# Autodesk Inventor assembly: SimpleDesignV2 - 02
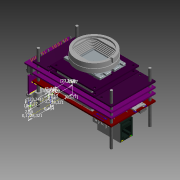
[picture p0: Inventor's stored thumbnail of the model, 180x180]
Saved by Autodesk Inventor 2015 (Build 190159000, 159)
## iProperties
Created: 2014-04-13
Part Number: SimpleDesignV2 - 02
Document SubType Name: Assembly
Designer: spichelh
Author: spichelh
## Documents named in this file (23)
- C:\Users\spichelh\Documents\GitHub\beta-hardware\Enclosure\SimpleDesign02\SimpleDesignV2 - 02.iam
- C:\Users\spichelh\Documents\GitHub\beta-hardware\Enclosure\SimpleDesign02\SFE-Host01.ipt
- C:\Users\spichelh\Documents\GitHub\beta-hardware\Enclosure\SimpleDesign02\SFE-ProcessingBoard01.ipt
- C:\Users\spichelh\Documents\GitHub\beta-hardware\Enclosure\SimpleDesign02\PCBModuleLeft02.ipt
- C:\Users\spichelh\Documents\GitHub\beta-hardware\Enclosure\SimpleDesign02\BetaBoard01.ipt
- C:\Users\spichelh\Documents\GitHub\beta-hardware\Enclosure\SimpleDesign02\PowerPCB01.ipt
- C:\Users\spichelh\Documents\GitHub\beta-hardware\Enclosure\SimpleDesign02\Samtec-PCIE-036-02-D-F-TH.ipt
- C:\Users\spichelh\Documents\GitHub\beta-hardware\Enclosure\SimpleDesign02\SensorCooler01.ipt
- C:\Users\spichelh\Documents\GitHub\beta-hardware\Enclosure\SimpleDesign02\CMV12000v1.ipt
- C:\Users\spichelh\Documents\GitHub\beta-hardware\Enclosure\SimpleDesign02\threaded-rod01.ipt
- C:\Users\spichelh\Documents\GitHub\beta-hardware\Enclosure\SimpleDesign02\Simple3DPrintEnclosure01.ipt
- C:\Users\spichelh\Documents\Inventor\Content Center Files\R2015\en-US\ANSI B18.6.4(04)\ANSI B18.6.4 - 4-24 - 0,375(1) B IA.ipt
- C:\Users\spichelh\Documents\GitHub\beta-hardware\Enclosure\SimpleDesign02\Simple3DPrintBackplate01.ipt
- C:\Users\spichelh\Documents\Inventor\Content Center Files\R2015\en-US\Nut GB_T 17880.1-1999\Nut GB_T 17880.1-1999 M3 x 7.5.ipt
- C:\Users\spichelh\Documents\GitHub\beta-hardware\Enclosure\SimpleDesign02\CoolingFan50x50-V01.ipt
- C:\Users\spichelh\Documents\Inventor\Content Center Files\R2015\en-US\ANSI B18.6.3(00)\ANSI B18.6.3 - 4-40 UNC - 0,125(32).ipt
- C:\Users\spichelh\Documents\GitHub\beta-hardware\Enclosure\SimpleDesign02\Sensormount_CMV12000.iam
- C:\Users\spichelh\Documents\GitHub\beta-hardware\Enclosure\SimpleDesign02\Sensormount_CMV12000_CNC.ipt
- C:\Users\spichelh\Documents\GitHub\beta-hardware\Enclosure\SimpleDesign02\footplate.ipt
- C:\Users\spichelh\Documents\GitHub\beta-hardware\Enclosure\SimpleDesign02\E Mount.ipt
- C:\Users\spichelh\Documents\GitHub\beta-hardware\Enclosure\SimpleDesign02\HDMI Plugin Module.ipt
- C:\Users\spichelh\Documents\GitHub\beta-hardware\Enclosure\SimpleDesign02\HDMIPluginModuleHolder02.ipt
- C:\Users\spichelh\Documents\GitHub\beta-hardware\Enclosure\SimpleDesign02\Zynq_Z010_uZed_F_Prod_simplified.ipt
## Components (37 placed, 22 different names)
1. SFE-Host01:1 — Mate:73, Flush:48, Flush:49, Flush:125, Flush:126, Mate:163
2. SFE-ProcessingBoard01:1 — Mate:73, Flush:48, Flush:49, Flush:109, Mate:134, Flush:112, Mate:136, Flush:123, Flush:124, Mate:159, Mate:209
3. PCBModuleLeft02:1 — Flush:109, Mate:134, Flush:113, Flush:114
4. BetaBoard01:1 — Mate:135, Flush:110, Flush:111, Flush:112, Mate:136, Flush:113, Flush:114, Mate:137, Mate:138, Flush:116, Mate:142, Mate:143, Flush:117, Mate:209
5. Zynq_Z010_uZed_F_Prod_simplified:1 — Mate:131, Flush:107, Flush:108, Mate:192, Mate:193, Mate:194, Mate:218
6. PowerPCB01:1 — Mate:131, Flush:107, Flush:108, Mate:135, Flush:110, Flush:111
7. Samtec-PCIE-036-02-D-F-TH:1 — Mate:137, Mate:138, Flush:116, Mate:219, Mate:221, Mate:222
8. Samtec-PCIE-036-02-D-F-TH:2 — Mate:142, Mate:143, Flush:117, Mate:213, Mate:214, Mate:215
9. SensorCooler01:1
10. PCBModuleLeft02:2 — Flush:123, Flush:124, Mate:159
11. CMV12000v1:1 — Flush:125, Flush:126, Mate:163, Mate:195, Flush:138, Mate:200, Mate:201
12. Sensormount_CMV12000_CNC:1 — Mate:195, Mate:196, Flush:137, Flush:138, Flush:139, Mate:197, Mate:198, Flush:140, Flush:141, Mate:199, Mate:200, Mate:201, Mate:202, Mate:203, Mate:204, Mate:205, Flush:146, Mate:206, Mate:208
13. threaded-rod01:1 — Mate:198, Flush:140
14. threaded-rod01:2 — Flush:139, Mate:197, Mate:217
15. threaded-rod01:3 — Mate:196, Flush:137, Mate:216
16. threaded-rod01:4 — Mate:177, Flush:141, Mate:199
17. Simple3DPrintEnclosure01:1 — Mate:173, Mate:174, Mate:175, Mate:176, Mate:185, Mate:186, Mate:187, Flush:133, Flush:134, Flush:135, Flush:136, Mate:202, Mate:203, Mate:204, Flush:142, Flush:143, Flush:144, Flush:145, Mate:210, Mate:211, Mate:212
18. Simple3DPrintBackplate01:1 — Mate:210, Mate:211, Mate:212
19. Cross Recessed 100° Flat Countersunk Head Tapping Screw - Type B - Type IA - Inch No. 4 - 24 -  3/8:1 — Mate:173, Flush:143
20. Cross Recessed 100° Flat Countersunk Head Tapping Screw - Type B - Type IA - Inch No. 4 - 24 -  3/8:2 — Mate:174, Flush:142
21. Cross Recessed 100° Flat Countersunk Head Tapping Screw - Type B - Type IA - Inch No. 4 - 24 -  3/8:3 — Mate:175, Flush:145
22. Cross Recessed 100° Flat Countersunk Head Tapping Screw - Type B - Type IA - Inch No. 4 - 24 -  3/8:4 — Mate:176, Flush:144
23. Nut GB/T 17880.1-1999 M3 x 7.5:1 — Mate:177
24. Nut GB/T 17880.1-1999 M3 x 7.5:2
25. Nut GB/T 17880.1-1999 M3 x 7.5:3
26. Nut GB/T 17880.1-1999 M3 x 7.5:4
27. CoolingFan50x50-V01:1 — Mate:185, Mate:186, Mate:187, Mate:188, Mate:189, Mate:190, Mate:191
28. Cross Recessed 100° Flat Countersunk Head Machine Screw - Type I - Inch 4-40 UNC x 0,125:1 — Mate:188, Flush:135
29. Cross Recessed 100° Flat Countersunk Head Machine Screw - Type I - Inch 4-40 UNC x 0,125:2 — Mate:189, Flush:133
30. Cross Recessed 100° Flat Countersunk Head Machine Screw - Type I - Inch 4-40 UNC x 0,125:3 — Mate:190, Flush:134
31. Cross Recessed 100° Flat Countersunk Head Machine Screw - Type I - Inch 4-40 UNC x 0,125:4 — Mate:191, Flush:136
32. Heatsink 31x31x10mm [sub-assembly] — Mate:192, Mate:193, Mate:194
33. footplate:1 — Mate:205, Flush:146, Mate:206, Mate:207
34. E Mount:1 — Mate:208
35. HDMIPluginModuleHolder02:1 — Mate:216, Mate:217, Mate:218
36. HDMI Plugin Module:1 — Mate:213, Mate:214, Mate:215
37. HDMI Plugin Module:2 — Mate:219, Mate:221, Mate:222
## Relationships (83: Mate 53, Flush 30)
- Mate:73: SFE-Host01:1 ↔ SFE-ProcessingBoard01:1
- Flush:48: SFE-Host01:1 ↔ SFE-ProcessingBoard01:1
- Flush:49: SFE-Host01:1 ↔ SFE-ProcessingBoard01:1
- Mate:131 (7 mm): Zynq_Z010_uZed_F_Prod_simplified:1 ↔ PowerPCB01:1
- Flush:107: Zynq_Z010_uZed_F_Prod_simplified:1 ↔ PowerPCB01:1
- Flush:108: Zynq_Z010_uZed_F_Prod_simplified:1 ↔ PowerPCB01:1
- Flush:109: SFE-ProcessingBoard01:1 ↔ PCBModuleLeft02:1
- Mate:134 (1 mm): SFE-ProcessingBoard01:1 ↔ PCBModuleLeft02:1
- Mate:135 (5 mm): BetaBoard01:1 ↔ PowerPCB01:1
- Flush:110: BetaBoard01:1 ↔ PowerPCB01:1
- Flush:111: BetaBoard01:1 ↔ PowerPCB01:1
- Flush:112: SFE-ProcessingBoard01:1 ↔ BetaBoard01:1
- Mate:136: SFE-ProcessingBoard01:1 ↔ BetaBoard01:1
- Flush:113: PCBModuleLeft02:1 ↔ BetaBoard01:1
- Flush:114: PCBModuleLeft02:1 ↔ BetaBoard01:1
- Mate:137: BetaBoard01:1 ↔ Samtec-PCIE-036-02-D-F-TH:1
- Mate:138: BetaBoard01:1 ↔ Samtec-PCIE-036-02-D-F-TH:1
- Flush:116 (1.4908 mm): BetaBoard01:1 ↔ Samtec-PCIE-036-02-D-F-TH:1
- Mate:142: BetaBoard01:1 ↔ Samtec-PCIE-036-02-D-F-TH:2
- Mate:143: BetaBoard01:1 ↔ Samtec-PCIE-036-02-D-F-TH:2
- Flush:117 (2.0906 mm): BetaBoard01:1 ↔ Samtec-PCIE-036-02-D-F-TH:2
- Flush:123: SFE-ProcessingBoard01:1 ↔ PCBModuleLeft02:2
- Flush:124: SFE-ProcessingBoard01:1 ↔ PCBModuleLeft02:2
- Mate:159 (2 mm): SFE-ProcessingBoard01:1 ↔ PCBModuleLeft02:2
- Flush:125 (11.875 mm): SFE-Host01:1 ↔ CMV12000v1:1
- Flush:126 (5.175 mm): SFE-Host01:1 ↔ CMV12000v1:1
- Mate:163 (3 mm): SFE-Host01:1 ↔ CMV12000v1:1
- Mate:173: Simple3DPrintEnclosure01:1 ↔ Cross Recessed 100° Flat Countersunk Head Tapping Screw - Type B - Type IA - Inch No. 4 - 24 -  3/8:1
- Mate:174: Simple3DPrintEnclosure01:1 ↔ Cross Recessed 100° Flat Countersunk Head Tapping Screw - Type B - Type IA - Inch No. 4 - 24 -  3/8:2
- Mate:175: Simple3DPrintEnclosure01:1 ↔ Cross Recessed 100° Flat Countersunk Head Tapping Screw - Type B - Type IA - Inch No. 4 - 24 -  3/8:3
- Mate:176: Simple3DPrintEnclosure01:1 ↔ Cross Recessed 100° Flat Countersunk Head Tapping Screw - Type B - Type IA - Inch No. 4 - 24 -  3/8:4
- Mate:177: threaded-rod01:4 ↔ Nut GB/T 17880.1-1999 M3 x 7.5:1
- Mate:185: Simple3DPrintEnclosure01:1 ↔ CoolingFan50x50-V01:1
- Mate:186: Simple3DPrintEnclosure01:1 ↔ CoolingFan50x50-V01:1
- Mate:187: Simple3DPrintEnclosure01:1 ↔ CoolingFan50x50-V01:1
- Mate:188: CoolingFan50x50-V01:1 ↔ Cross Recessed 100° Flat Countersunk Head Machine Screw - Type I - Inch 4-40 UNC x 0,125:1
- Mate:189: CoolingFan50x50-V01:1 ↔ Cross Recessed 100° Flat Countersunk Head Machine Screw - Type I - Inch 4-40 UNC x 0,125:2
- Mate:190: CoolingFan50x50-V01:1 ↔ Cross Recessed 100° Flat Countersunk Head Machine Screw - Type I - Inch 4-40 UNC x 0,125:3
- Mate:191: CoolingFan50x50-V01:1 ↔ Cross Recessed 100° Flat Countersunk Head Machine Screw - Type I - Inch 4-40 UNC x 0,125:4
- Flush:133: Simple3DPrintEnclosure01:1 ↔ Cross Recessed 100° Flat Countersunk Head Machine Screw - Type I - Inch 4-40 UNC x 0,125:2
- Flush:134: Simple3DPrintEnclosure01:1 ↔ Cross Recessed 100° Flat Countersunk Head Machine Screw - Type I - Inch 4-40 UNC x 0,125:3
- Flush:135: Simple3DPrintEnclosure01:1 ↔ Cross Recessed 100° Flat Countersunk Head Machine Screw - Type I - Inch 4-40 UNC x 0,125:1
- Flush:136: Simple3DPrintEnclosure01:1 ↔ Cross Recessed 100° Flat Countersunk Head Machine Screw - Type I - Inch 4-40 UNC x 0,125:4
- Mate:192: Zynq_Z010_uZed_F_Prod_simplified:1 ↔ Heatsink 31x31x10mm
- Mate:193 (2 mm): Zynq_Z010_uZed_F_Prod_simplified:1 ↔ Heatsink 31x31x10mm
- Mate:194 (3 mm): Zynq_Z010_uZed_F_Prod_simplified:1 ↔ Heatsink 31x31x10mm
- Mate:195: CMV12000v1:1 ↔ Sensormount_CMV12000_CNC:1
- Mate:196: Sensormount_CMV12000_CNC:1 ↔ threaded-rod01:3
- Flush:137: Sensormount_CMV12000_CNC:1 ↔ threaded-rod01:3
- Flush:138: CMV12000v1:1 ↔ Sensormount_CMV12000_CNC:1
- Flush:139: Sensormount_CMV12000_CNC:1 ↔ threaded-rod01:2
- Mate:197: Sensormount_CMV12000_CNC:1 ↔ threaded-rod01:2
- Mate:198: Sensormount_CMV12000_CNC:1 ↔ threaded-rod01:1
- Flush:140: Sensormount_CMV12000_CNC:1 ↔ threaded-rod01:1
- Flush:141: Sensormount_CMV12000_CNC:1 ↔ threaded-rod01:4
- Mate:199: Sensormount_CMV12000_CNC:1 ↔ threaded-rod01:4
- Mate:200 (0.1 mm): CMV12000v1:1 ↔ Sensormount_CMV12000_CNC:1
- Mate:201 (0.1 mm): CMV12000v1:1 ↔ Sensormount_CMV12000_CNC:1
- Mate:202: Sensormount_CMV12000_CNC:1 ↔ Simple3DPrintEnclosure01:1
- Mate:203: Sensormount_CMV12000_CNC:1 ↔ Simple3DPrintEnclosure01:1
- Mate:204: Sensormount_CMV12000_CNC:1 ↔ Simple3DPrintEnclosure01:1
- Flush:142: Simple3DPrintEnclosure01:1 ↔ Cross Recessed 100° Flat Countersunk Head Tapping Screw - Type B - Type IA - Inch No. 4 - 24 -  3/8:2
- Flush:143: Simple3DPrintEnclosure01:1 ↔ Cross Recessed 100° Flat Countersunk Head Tapping Screw - Type B - Type IA - Inch No. 4 - 24 -  3/8:1
- Flush:144: Simple3DPrintEnclosure01:1 ↔ Cross Recessed 100° Flat Countersunk Head Tapping Screw - Type B - Type IA - Inch No. 4 - 24 -  3/8:4
- Flush:145: Simple3DPrintEnclosure01:1 ↔ Cross Recessed 100° Flat Countersunk Head Tapping Screw - Type B - Type IA - Inch No. 4 - 24 -  3/8:3
- Mate:205: Sensormount_CMV12000_CNC:1 ↔ footplate:1
- Flush:146: Sensormount_CMV12000_CNC:1 ↔ footplate:1
- Mate:206 (13.575 mm): Sensormount_CMV12000_CNC:1 ↔ footplate:1
- Mate:207: footplate:1
- Mate:208: Sensormount_CMV12000_CNC:1 ↔ E Mount:1
- Mate:209 (5 mm): SFE-ProcessingBoard01:1 ↔ BetaBoard01:1
- Mate:210: Simple3DPrintEnclosure01:1 ↔ Simple3DPrintBackplate01:1
- Mate:211: Simple3DPrintEnclosure01:1 ↔ Simple3DPrintBackplate01:1
- Mate:212: Simple3DPrintEnclosure01:1 ↔ Simple3DPrintBackplate01:1
- Mate:213: Samtec-PCIE-036-02-D-F-TH:2 ↔ HDMI Plugin Module:1
- Mate:214: Samtec-PCIE-036-02-D-F-TH:2 ↔ HDMI Plugin Module:1
- Mate:215: Samtec-PCIE-036-02-D-F-TH:2 ↔ HDMI Plugin Module:1
- Mate:216: threaded-rod01:3 ↔ HDMIPluginModuleHolder02:1
- Mate:217: threaded-rod01:2 ↔ HDMIPluginModuleHolder02:1
- Mate:218 (15.525 mm): Zynq_Z010_uZed_F_Prod_simplified:1 ↔ HDMIPluginModuleHolder02:1
- Mate:219: Samtec-PCIE-036-02-D-F-TH:1 ↔ HDMI Plugin Module:2
- Mate:221: Samtec-PCIE-036-02-D-F-TH:1 ↔ HDMI Plugin Module:2
- Mate:222: Samtec-PCIE-036-02-D-F-TH:1 ↔ HDMI Plugin Module:2
